# Autodesk Inventor assembly: left wheel with clamping hub
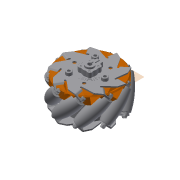
[picture p0: Inventor's stored thumbnail of the model, 180x180]
Saved by Autodesk Inventor 2018 (Build 220112000, 112)
## iProperties
Created: 2019-09-27
Part Number: left wheel with clamping hub
Document SubType Name: Assembly
Designer: ball
Author: ball
## Documents named in this file (3)
- C:\FTC\FTC8863CAD\2019 Robot\Mecanum Drive Train\left wheel with clamping hub.iam
- C:\FTC\FTC8863CAD\2019 Robot\Mecanum Drive Train\left wheel.iam
- C:\FTC\FTC8863CAD\Actobotics\545 parts\545618 assembly.ipt
## Components (3 placed, 2 different names)
1. left wheel:1 [sub-assembly] — Mate:2, Mate:4, Mate:5, Mate:6
2. 545618 assembly:1 — Mate:2, Flush:1, Mate:6
3. 545618 assembly:2 — Mate:4, Flush:1, Mate:5
## Relationships (5: Mate 4, Flush 1)
- Mate:2: left wheel:1 ↔ 545618 assembly:1
- Mate:4: left wheel:1 ↔ 545618 assembly:2
- Flush:1: 545618 assembly:1 ↔ 545618 assembly:2
- Mate:5: left wheel:1 ↔ 545618 assembly:2
- Mate:6: left wheel:1 ↔ 545618 assembly:1
